# Autodesk Inventor assembly: wheel tip assembly 2018 ver_MIR
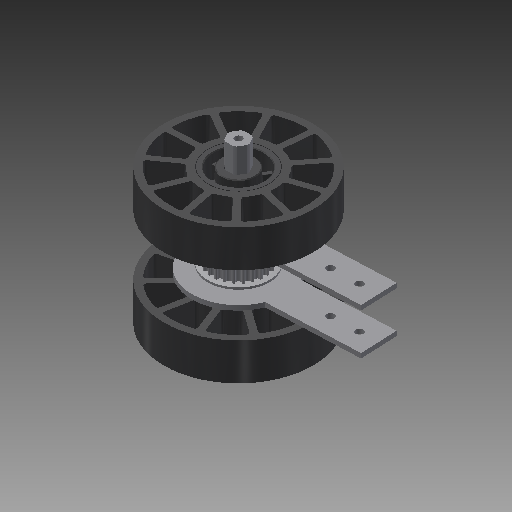
[picture p0: Inventor's stored thumbnail of the model, 512x512]
Saved by Autodesk Inventor 2018 (Build 220112000, 112)
## iProperties
Created: 2019-02-24
Part Number: wheel tip assembly 2018 ver_MIR
Document SubType Name: Assembly
Designer: Tiberus
Author: Tiberus
## Documents named in this file (6)
- C:\Users\Tiberus\Documents\GitHub\2019CAD\NEW NEW GRIPPER (feb 23)\wheel tip assembly 2018 ver_MIR.iam
- C:\Users\Tiberus\Documents\GitHub\2019CAD\NEW NEW GRIPPER (feb 23)\wheel tip_MIR.ipt
- C:\Users\Tiberus\Documents\GitHub\2019CAD\NEW NEW GRIPPER (feb 23)\0_500_ID_x_1_125_OD_x_0_313_WD_Flanged_Bearing_217-2731_MIR.ipt
- C:\Users\Tiberus\Documents\GitHub\2019CAD\NEW NEW GRIPPER (feb 23)\1_2_Hex_x_0_201_ID_ThunderHex_Stock_18_217-4002_MIR.ipt
- C:\Users\Tiberus\Documents\GitHub\2019CAD\NEW NEW GRIPPER (feb 23)\am-3480 4IN 500Hex Bore Compliant Wheel_MIR.ipt
- C:\Users\Tiberus\Documents\GitHub\2019CAD\NEW NEW GRIPPER (feb 23)\24t_x_15mm_Wide_Aluminum_Pulley_HTD_5mm_1_2_Hex_217-4101_MIR.ipt
## Components (8 placed, 5 different names)
1. wheel tip_MIR:1 — Flush:2, Flush:1, Mate:4, Mate:3
2. wheel tip_MIR:2 — Flush:2, Flush:1, Mate:2, Mate:1
3. 0_500_ID_x_1_125_OD_x_0_313_WD_Flanged_Bearing_217-2731_MIR:1 — Mate:2, Mate:1, Mate:10, Mate:14
4. 0_500_ID_x_1_125_OD_x_0_313_WD_Flanged_Bearing_217-2731_MIR:2 — Mate:4, Mate:3, Mate:9, Mate:13
5. 1_2_Hex_x_0_201_ID_ThunderHex_Stock_18_217-4002_MIR:1 — Mate:10, Mate:9, Mate:8, Mate:7, Mate:6, Mate:5, Mate:12, Mate:11
6. am-3480 4IN 500Hex Bore Compliant Wheel_MIR:1 — Mate:8, Mate:7
7. am-3480 4IN 500Hex Bore Compliant Wheel_MIR:2 — Mate:6, Mate:5
8. 24t_x_15mm_Wide_Aluminum_Pulley_HTD_5mm_1_2_Hex_217-4101_MIR:1 — Mate:14, Mate:13, Mate:12, Mate:11
## Relationships (16: Mate 14, Flush 2)
- Flush:2: wheel tip_MIR:1 ↔ wheel tip_MIR:2
- Flush:1: wheel tip_MIR:1 ↔ wheel tip_MIR:2
- Mate:2: wheel tip_MIR:2 ↔ 0_500_ID_x_1_125_OD_x_0_313_WD_Flanged_Bearing_217-2731_MIR:1
- Mate:1: wheel tip_MIR:2 ↔ 0_500_ID_x_1_125_OD_x_0_313_WD_Flanged_Bearing_217-2731_MIR:1
- Mate:4: wheel tip_MIR:1 ↔ 0_500_ID_x_1_125_OD_x_0_313_WD_Flanged_Bearing_217-2731_MIR:2
- Mate:3: wheel tip_MIR:1 ↔ 0_500_ID_x_1_125_OD_x_0_313_WD_Flanged_Bearing_217-2731_MIR:2
- Mate:10: 0_500_ID_x_1_125_OD_x_0_313_WD_Flanged_Bearing_217-2731_MIR:1 ↔ 1_2_Hex_x_0_201_ID_ThunderHex_Stock_18_217-4002_MIR:1
- Mate:9: 0_500_ID_x_1_125_OD_x_0_313_WD_Flanged_Bearing_217-2731_MIR:2 ↔ 1_2_Hex_x_0_201_ID_ThunderHex_Stock_18_217-4002_MIR:1
- Mate:8: 1_2_Hex_x_0_201_ID_ThunderHex_Stock_18_217-4002_MIR:1 ↔ am-3480 4IN 500Hex Bore Compliant Wheel_MIR:1
- Mate:7: 1_2_Hex_x_0_201_ID_ThunderHex_Stock_18_217-4002_MIR:1 ↔ am-3480 4IN 500Hex Bore Compliant Wheel_MIR:1
- Mate:6: 1_2_Hex_x_0_201_ID_ThunderHex_Stock_18_217-4002_MIR:1 ↔ am-3480 4IN 500Hex Bore Compliant Wheel_MIR:2
- Mate:5: 1_2_Hex_x_0_201_ID_ThunderHex_Stock_18_217-4002_MIR:1 ↔ am-3480 4IN 500Hex Bore Compliant Wheel_MIR:2
- Mate:14: 0_500_ID_x_1_125_OD_x_0_313_WD_Flanged_Bearing_217-2731_MIR:1 ↔ 24t_x_15mm_Wide_Aluminum_Pulley_HTD_5mm_1_2_Hex_217-4101_MIR:1
- Mate:13: 0_500_ID_x_1_125_OD_x_0_313_WD_Flanged_Bearing_217-2731_MIR:2 ↔ 24t_x_15mm_Wide_Aluminum_Pulley_HTD_5mm_1_2_Hex_217-4101_MIR:1
- Mate:12: 1_2_Hex_x_0_201_ID_ThunderHex_Stock_18_217-4002_MIR:1 ↔ 24t_x_15mm_Wide_Aluminum_Pulley_HTD_5mm_1_2_Hex_217-4101_MIR:1
- Mate:11: 1_2_Hex_x_0_201_ID_ThunderHex_Stock_18_217-4002_MIR:1 ↔ 24t_x_15mm_Wide_Aluminum_Pulley_HTD_5mm_1_2_Hex_217-4101_MIR:1
